# Autodesk Inventor assembly: back_assembly
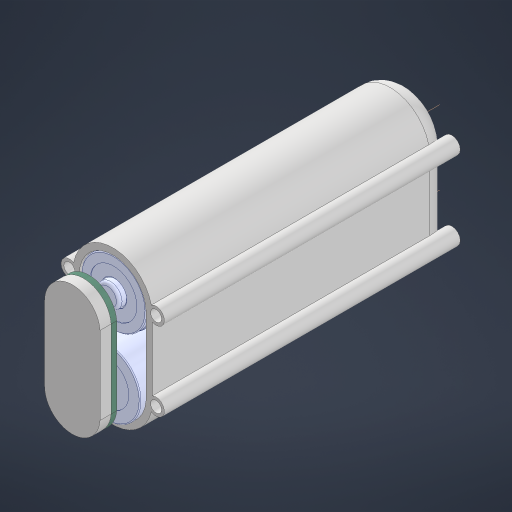
[picture p0: Inventor's stored thumbnail of the model, 512x512]
Saved by Autodesk Inventor 2024 (Build 280153000, 153)
## iProperties
Created: 2026-08-20
Part Number: back_assembly
Document SubType Name: Assembly
Designer: schar
Author: schar
## Documents named in this file (5)
- C:\Users\schar\Projects\SpeleoFox\cad\Speleofox PCB\back_assembly.iam
- C:\Users\schar\Projects\SpeleoFox\cad\Speleofox PCB\BAT_speleopcb_part.ipt
- C:\Users\schar\Projects\SpeleoFox\cad\assets\18650 Battery.ipt
- C:\Users\schar\Projects\SpeleoFox\cad\assets\battery_case_shell.ipt
- C:\Users\schar\Projects\SpeleoFox\cad\Speleofox PCB\battery_case_top.ipt
## Components (6 placed, 4 different names)
1. BAT_speleopcb_part:1 — Mate:1, Mate:2, Flush:1, Flush:2, Flush:3
2. 18650 Battery:1 — Mate:1, Mate:3
3. 18650 Battery:2 — Mate:2, Mate:4, Mate:11
4. battery_case_shell:1 — Flush:1, Flush:2, Flush:3, Mate:5, Mate:6, Mate:9, Mate:10
5. BAT_speleopcb_part:2 — Mate:7, Mate:8, Mate:11, Flush:4, Flush:5, Flush:6
6. battery_case_top:1 — Flush:4, Flush:5, Flush:6
## Relationships (17: Mate 11, Flush 6)
- Mate:1 (5 mm): BAT_speleopcb_part:1 ↔ 18650 Battery:1
- Mate:2 (5 mm): BAT_speleopcb_part:1 ↔ 18650 Battery:2
- Flush:1: BAT_speleopcb_part:1 ↔ battery_case_shell:1
- Flush:2: BAT_speleopcb_part:1 ↔ battery_case_shell:1
- Flush:3: BAT_speleopcb_part:1 ↔ battery_case_shell:1
- Mate:3: 18650 Battery:1
- Mate:4: 18650 Battery:2
- Mate:5: battery_case_shell:1
- Mate:6: battery_case_shell:1
- Mate:7: BAT_speleopcb_part:2
- Mate:8: BAT_speleopcb_part:2
- Mate:9: battery_case_shell:1
- Mate:10: battery_case_shell:1
- Mate:11 (5 mm): 18650 Battery:2 ↔ BAT_speleopcb_part:2
- Flush:4: BAT_speleopcb_part:2 ↔ battery_case_top:1
- Flush:5: BAT_speleopcb_part:2 ↔ battery_case_top:1
- Flush:6: BAT_speleopcb_part:2 ↔ battery_case_top:1
